# Autodesk Inventor assembly: main gripper assembly
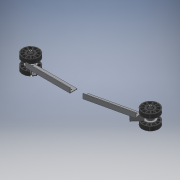
[picture p0: Inventor's stored thumbnail of the model, 180x180]
Saved by Autodesk Inventor 2018 (Build 220112000, 112)
## iProperties
Created: 2019-02-23
Part Number: main gripper assembly
Document SubType Name: Assembly
Designer: s-2513225
Author: s-2513225
## Documents named in this file (5)
- C:\Users\s-2513225\Downloads\2019CAD-master\NEW NEW GRIPPER (feb 23)\main gripper assembly.iam
- C:\Users\s-2513225\Downloads\2019CAD-master\NEW NEW GRIPPER (feb 23)\wheel tip assembly.iam
- C:\Users\s-2513225\Downloads\2019CAD-master\NEW NEW GRIPPER (feb 23)\wheel tip connector 1.ipt
- C:\Users\s-2513225\Downloads\2019CAD-master\NEW NEW GRIPPER (feb 23)\angle iron with  holes 1.ipt
- C:\Users\s-2513225\Downloads\2019CAD-master\NEW NEW GRIPPER (feb 23)\angle iron with  holes 2.ipt
## Components (6 placed, 4 different names)
1. wheel tip assembly:1 [sub-assembly] — Mate:4, Mate:5, Mate:6, Mate:11, Mate:13
2. wheel tip connector 1:1 — Mate:4, Mate:5, Mate:6, Mate:12
3. wheel tip assembly:2 [sub-assembly] — Mate:1, Mate:2, Mate:3, Mate:8, Mate:9, Mate:10
4. wheel tip connector 1:2 — Mate:1, Mate:2, Mate:3
5. angle iron with  holes 1:1 — Mate:8, Mate:9, Mate:10
6. angle iron with  holes 2:1 — Mate:11, Mate:12, Mate:13
## Relationships (12: Mate 12)
- Mate:1: wheel tip assembly:2 ↔ wheel tip connector 1:2
- Mate:2: wheel tip assembly:2 ↔ wheel tip connector 1:2
- Mate:3: wheel tip assembly:2 ↔ wheel tip connector 1:2
- Mate:4: wheel tip assembly:1 ↔ wheel tip connector 1:1
- Mate:5: wheel tip assembly:1 ↔ wheel tip connector 1:1
- Mate:6: wheel tip assembly:1 ↔ wheel tip connector 1:1
- Mate:8: wheel tip assembly:2 ↔ angle iron with  holes 1:1
- Mate:9: wheel tip assembly:2 ↔ angle iron with  holes 1:1
- Mate:10: wheel tip assembly:2 ↔ angle iron with  holes 1:1
- Mate:11: wheel tip assembly:1 ↔ angle iron with  holes 2:1
- Mate:12: wheel tip connector 1:1 ↔ angle iron with  holes 2:1
- Mate:13: wheel tip assembly:1 ↔ angle iron with  holes 2:1
